# Autodesk Inventor assembly: Manija completa
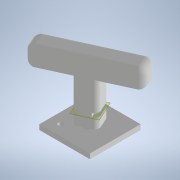
[picture p0: Inventor's stored thumbnail of the model, 180x180]
Saved by Autodesk Inventor 2020.3 (Build 243373000, 373)
## iProperties
Created: 2020-08-22
Part Number: Manija completa
Document SubType Name: Assembly
Designer: miosh
Author: miosh
## Documents named in this file (3)
- D:\Archivos Carlos\Archivos Inventor\Manija completa.iam
- D:\Archivos Carlos\Archivos Inventor\Base Manija.ipt
- D:\Archivos Carlos\Archivos Inventor\Manija.ipt
## Components (2 placed, 2 different names)
1. Base Manija:1 — Insertar:1
2. Manija:1 — Insertar:1
## Relationships (1: Insert 1)
- Insertar:1: Base Manija:1 ↔ Manija:1
